# Autodesk Inventor assembly: 揺動節+ヘッケン_MIR
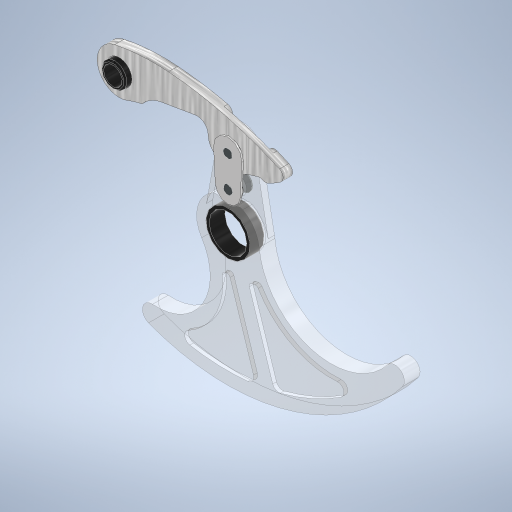
[picture p0: Inventor's stored thumbnail of the model, 512x512]
Saved by Autodesk Inventor 2023 (Build 270158000, 158)
## iProperties
Created: 2022-01-08
Part Number: 揺動節+ヘッケン_MIR
Document SubType Name: Assembly
Designer: muzho
Mass: 17.1342 g
Surface Area: 87.451 cm^2
Volume: 10.1847 cm^3
Density: 1.68235 g/cm^3
Author: acps
## Documents named in this file (8)
- C:\Users\muzho\Documents\srdc\srdc_2\脚\MIR\揺動節+ヘッケン_MIR.iam
- C:\Users\muzho\Documents\srdc\srdc_2\脚\MIR\揺動節_MIR.ipt
- C:\Users\muzho\Documents\srdc\srdc_2\脚\MIR\ヘッケン_MIR.ipt
- C:\Users\muzho\Documents\srdc\srdc_2\脚\MIR\ヘッケン抑え_MIR.ipt
- C:\Users\muzho\Documents\srdc\srdc_2\オイレス\MIR\w5f12-14n_MIR.ipt
- C:\Users\muzho\Documents\srdc\srdc_2\オイレス\MIR\w1.5f5-7n_MIR.ipt
- C:\Users\muzho\Documents\srdc\srdc_2\オイレス\MIR\w5f6-12a_MIR.ipt
- C:\Users\muzho\Documents\srdc\srdc_2\ねじ\MIR\m3皿ネジ5_MIR.ipt
## Components (8 placed, 7 different names)
1. 揺動節_MIR:1 — 挿入:6, 挿入:5
2. ヘッケン_MIR:1 — 挿入:6, 挿入:8, メイト:2, メイト:1, 挿入:9, 挿入:7, 挿入:10, 挿入:11
3. ヘッケン抑え_MIR:1 — 挿入:8, メイト:2, メイト:1
4. w5f12-14n_MIR:1 — 挿入:9
5. w1.5f5-7n_MIR:1 — 挿入:7
6. w5f6-12a_MIR:1 — 挿入:5
7. m3皿ネジ5_MIR:1 — 挿入:10
8. m3皿ネジ5_MIR:2 — 挿入:11
## Relationships (9: Insert 7, Mate 2)
- 挿入:6 [Insert]: 揺動節_MIR:1 ↔ ヘッケン_MIR:1
- 挿入:8 [Insert]: ヘッケン_MIR:1 ↔ ヘッケン抑え_MIR:1
- メイト:2 [Mate]: ヘッケン_MIR:1 ↔ ヘッケン抑え_MIR:1
- メイト:1 [Mate]: ヘッケン_MIR:1 ↔ ヘッケン抑え_MIR:1
- 挿入:9 [Insert]: ヘッケン_MIR:1 ↔ w5f12-14n_MIR:1
- 挿入:7 [Insert]: ヘッケン_MIR:1 ↔ w1.5f5-7n_MIR:1
- 挿入:5 [Insert]: 揺動節_MIR:1 ↔ w5f6-12a_MIR:1
- 挿入:10 [Insert]: ヘッケン_MIR:1 ↔ m3皿ネジ5_MIR:1
- 挿入:11 [Insert]: ヘッケン_MIR:1 ↔ m3皿ネジ5_MIR:2
